# Autodesk Inventor assembly: Electronics V2
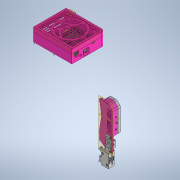
[picture p0: Inventor's stored thumbnail of the model, 180x180]
Saved by Autodesk Inventor 2020.3 (Build 243373010, 373A)
## iProperties
Created: 2019-12-13
Part Number: Electronics V2
Document SubType Name: Assembly
Designer: pepd9
Mass: 362.795 g
Surface Area: 2325.02 cm^2
Volume: 298.236 cm^3
Density: 1.21647 g/cm^3
Author: pepd9
## Documents named in this file (19)
- D:\Designs\MK3PRO P1\ELECTRONICS\Electronics V2.iam
- D:\Designs\MK3PRO P1\COMPONENTS\SHCS_M3_12.ipt
- D:\Designs\MK3PRO P1\COMPONENTS\M3 Nut.ipt
- D:\Designs\MK3PRO P1\ELECTRONICS\LM2596.ipt
- D:\Designs\MK3PRO P1\ELECTRONICS\FAN PS CASE.ipt
- D:\Designs\MK3PRO P1\COMPONENTS\SHCS_M3_8.ipt
- D:\Designs\MK3PRO P1\COMPONENTS\NUT_SQUARE_M3.ipt
- D:\Designs\MK3PRO P1\COMPONENTS\SHCS_M3_10.ipt
- D:\Designs\MK3PRO P1\ELECTRONICS\FAN PS CASE LID.ipt
- D:\Designs\MK3PRO P1\ELECTRONICS\Fan Distribution Case.ipt
- D:\Designs\MK3PRO P1\ELECTRONICS\Double Sided PCB 6x28.iam
- D:\Designs\MK3PRO P1\COMPONENTS\M3 Washer.ipt
- D:\Designs\MK3PRO P1\FRAME\Extruder-Motherboard Cable Clamp.ipt
- D:\Designs\MK3PRO P1\COMPONENTS\SHCS_M3_20.ipt
- D:\Designs\MK3PRO P1\ELECTRONICS\Fan PDP Lid.ipt
- D:\Designs\MK3PRO P1\ELECTRONICS\ID Plate.ipt
- D:\Designs\MK3PRO P1\ELECTRONICS\Rambo Case P1.0.ipt
- D:\Designs\MK3PRO P1\ELECTRONICS\Rambo 1.3.ipt
- D:\Designs\MK3PRO P1\ELECTRONICS\Rambo Case Lid.ipt
## Components (56 placed, 18 different names)
1. LM2596:1 — Mate:14, Mate:15, Mate:18, Mate:19, Mate:20
2. FAN PS CASE:1 — Mate:14, Mate:15, Mate:16, Mate:17, Mate:20, Mate:21, Mate:22, Angle:6, Angle:7, Mate:25, Mate:26, Angle:8, Mate:27, Mate:28, Mate:29, Mate:30, Mate:31, Mate:32, Angle:9
3. SHCS_M3_8:1 — Mate:17, Mate:19, Mate:24
4. SHCS_M3_8:2 — Mate:16, Mate:18, Mate:23
5. M3 Nut:5 — Mate:21, Angle:7, Mate:24
6. M3 Nut:6 — Mate:22, Angle:6, Mate:23
7. NUT_SQUARE_M3:1 — Mate:25, Mate:26, Angle:8
8. SHCS_M3_10:1 — Mate:28, Mate:29
9. SHCS_M3_10:2 — Mate:27, Mate:30
10. SHCS_M3_8:3 — Mate:33, Mate:34
11. FAN PS CASE LID:1 — Mate:31, Mate:32, Angle:9, Mate:33, Mate:34
12. Fan Distribution Case:1 — Mate:35, Angle:10, Mate:36, Mate:37, Mate:42, Mate:44, Mate:47, Mate:56, Mate:57, Mate:58, Mate:59, Angle:11, Angle:12, Mate:64, Mate:65, Mate:66, Mate:67, Mate:72, Mate:73, Mate:74, Mate:75, Angle:15, Angle:16, Mate:76, Mate:77, Mate:84, Angle:17, Mate:86, Angle:18, Mate:138, Mate:139, Mate:140, Mate:142, Mate:147, Flush:1, Mate:149
13. Double Sided PCB 6x28:1 [sub-assembly] — Mate:35, Angle:10, Mate:36, Mate:37
14. Extruder-Motherboard Cable Clamp:2 — Mate:42, Mate:44, Mate:47, Mate:48, Mate:49, Mate:52, Mate:53
15. SHCS_M3_20:2 — Mate:49, Mate:53, Mate:62
16. SHCS_M3_20:4 — Mate:48, Mate:52, Mate:63
17. M3 Nut:7 — Mate:59
18. M3 Nut:8 — Mate:58
19. M3 Nut:9 — Mate:57, Mate:62, Angle:12
20. M3 Nut:10 — Mate:56, Mate:63, Angle:11
21. M3 Nut:11 — Mate:73, Mate:74, Angle:15
22. M3 Nut:12 — Mate:72, Mate:75, Angle:16
23. M3 Washer:2 — Mate:64, Mate:69, Mate:70
24. M3 Washer:3 — Mate:65, Mate:68, Mate:71
25. SHCS_M3_10:4 — Mate:66, Mate:69, Mate:70
26. SHCS_M3_10:5 — Mate:67, Mate:68, Mate:71
27. SHCS_M3_8:4 — Mate:76, Mate:144, Mate:145
28. SHCS_M3_8:5 — Mate:77, Mate:143, Mate:146
29. SHCS_M3_12:3 — Mate:87, Mate:148, Mate:163
30. SHCS_M3_12:4 — Mate:85
31. NUT_SQUARE_M3:2 — Mate:84, Mate:85, Angle:17
32. NUT_SQUARE_M3:3 — Mate:86, Mate:87, Angle:18
33. Rambo Case P1.0:1 — Mate:88, Mate:89, Mate:90, Mate:113, Mate:114, Mate:115, Mate:116, Mate:117, Mate:118, Mate:119, Mate:120, Mate:121, Mate:122, Mate:123, Mate:124, Mate:125, Mate:126, Angle:24, Angle:25, Angle:26, Angle:27, Mate:137, Mate:150, Mate:151, Mate:152, Mate:153, Mate:154, Mate:156, Mate:159, Angle:28
34. Rambo 1.3:1 — Mate:88, Mate:89, Mate:90, Mate:129, Mate:130, Mate:131, Mate:132, Mate:133, Mate:134, Mate:135, Mate:136
35. Rambo Case Lid:1 — Mate:137, Mate:150, Mate:151, Mate:152, Mate:158, Mate:160, Mate:161, Mate:162
36. SHCS_M3_12:5 — Mate:117, Mate:127
37. SHCS_M3_12:6 — Mate:118, Mate:128
38. M3 Washer:4 — Mate:114, Mate:115, Mate:128
39. M3 Washer:5 — Mate:113, Mate:116, Mate:127
40. M3 Nut:13 — Mate:120, Mate:126, Angle:24
41. M3 Nut:14 — Mate:121, Mate:124, Angle:26
42. M3 Nut:15 — Mate:122, Mate:123, Angle:27
43. M3 Nut:16 — Mate:119, Mate:125, Angle:25
44. SHCS_M3_8:6 — Mate:129, Mate:134
45. SHCS_M3_8:7 — Mate:130, Mate:135
46. SHCS_M3_8:8 — Mate:131, Mate:136
47. SHCS_M3_8:9 — Mate:132, Mate:133
48. SHCS_M3_10:6 — Mate:140, Mate:141
49. M3 Washer:6 — Mate:138, Mate:139, Mate:141
50. ID Plate:1 — Mate:142, Mate:143, Mate:144, Mate:145, Mate:146
51. Fan PDP Lid:1 — Mate:147, Mate:148, Flush:1, Mate:149, Mate:163, Mate:164, Mate:165
52. NUT_SQUARE_M3:4 — Mate:156, Mate:159, Angle:28
53. NUT_SQUARE_M3:5 — Mate:153, Mate:154
54. SHCS_M3_10:7 — Mate:158, Mate:160
55. SHCS_M3_10:9 — Mate:161, Mate:162
56. SHCS_M3_12:7 — Mate:164, Mate:165
## Relationships (126: Mate 109, Angle 16, Flush 1)
- Mate:14: LM2596:1 ↔ FAN PS CASE:1
- Mate:15: LM2596:1 ↔ FAN PS CASE:1
- Mate:16: FAN PS CASE:1 ↔ SHCS_M3_8:2
- Mate:17: FAN PS CASE:1 ↔ SHCS_M3_8:1
- Mate:18: LM2596:1 ↔ SHCS_M3_8:2
- Mate:19: LM2596:1 ↔ SHCS_M3_8:1
- Mate:20: LM2596:1 ↔ FAN PS CASE:1
- Mate:21: FAN PS CASE:1 ↔ M3 Nut:5
- Mate:22: FAN PS CASE:1 ↔ M3 Nut:6
- Angle:6 (0 deg): FAN PS CASE:1 ↔ M3 Nut:6
- Mate:23: SHCS_M3_8:2 ↔ M3 Nut:6
- Angle:7 (0 deg): FAN PS CASE:1 ↔ M3 Nut:5
- Mate:24: SHCS_M3_8:1 ↔ M3 Nut:5
- Mate:25: FAN PS CASE:1 ↔ NUT_SQUARE_M3:1
- Mate:26: FAN PS CASE:1 ↔ NUT_SQUARE_M3:1
- Angle:8 (0 deg): FAN PS CASE:1 ↔ NUT_SQUARE_M3:1
- Mate:27: FAN PS CASE:1 ↔ SHCS_M3_10:2
- Mate:28: FAN PS CASE:1 ↔ SHCS_M3_10:1
- Mate:29: FAN PS CASE:1 ↔ SHCS_M3_10:1
- Mate:30: FAN PS CASE:1 ↔ SHCS_M3_10:2
- Mate:31: FAN PS CASE:1 ↔ FAN PS CASE LID:1
- Mate:32: FAN PS CASE:1 ↔ FAN PS CASE LID:1
- Angle:9 (180 deg): FAN PS CASE:1 ↔ FAN PS CASE LID:1
- Mate:33: SHCS_M3_8:3 ↔ FAN PS CASE LID:1
- Mate:34: SHCS_M3_8:3 ↔ FAN PS CASE LID:1
- Mate:35: Fan Distribution Case:1 ↔ Double Sided PCB 6x28:1
- Angle:10 (0 deg): Fan Distribution Case:1 ↔ Double Sided PCB 6x28:1
- Mate:36 (-40 mm): Fan Distribution Case:1 ↔ Double Sided PCB 6x28:1
- Mate:37 (0.3 mm): Fan Distribution Case:1 ↔ Double Sided PCB 6x28:1
- Mate:42: Fan Distribution Case:1 ↔ Extruder-Motherboard Cable Clamp:2
- Mate:44: Fan Distribution Case:1 ↔ Extruder-Motherboard Cable Clamp:2
- Mate:47: Fan Distribution Case:1 ↔ Extruder-Motherboard Cable Clamp:2
- Mate:48: Extruder-Motherboard Cable Clamp:2 ↔ SHCS_M3_20:4
- Mate:49: Extruder-Motherboard Cable Clamp:2 ↔ SHCS_M3_20:2
- Mate:52: Extruder-Motherboard Cable Clamp:2 ↔ SHCS_M3_20:4
- Mate:53: Extruder-Motherboard Cable Clamp:2 ↔ SHCS_M3_20:2
- Mate:56: Fan Distribution Case:1 ↔ M3 Nut:10
- Mate:57: Fan Distribution Case:1 ↔ M3 Nut:9
- Mate:58: Fan Distribution Case:1 ↔ M3 Nut:8
- Mate:59: Fan Distribution Case:1 ↔ M3 Nut:7
- Mate:62: SHCS_M3_20:2 ↔ M3 Nut:9
- Mate:63: SHCS_M3_20:4 ↔ M3 Nut:10
- Angle:11 (0 deg): Fan Distribution Case:1 ↔ M3 Nut:10
- Angle:12 (0 deg): Fan Distribution Case:1 ↔ M3 Nut:9
- Mate:64: Fan Distribution Case:1 ↔ M3 Washer:2
- Mate:65: Fan Distribution Case:1 ↔ M3 Washer:3
- Mate:66: Fan Distribution Case:1 ↔ SHCS_M3_10:4
- Mate:67: Fan Distribution Case:1 ↔ SHCS_M3_10:5
- Mate:68: M3 Washer:3 ↔ SHCS_M3_10:5
- Mate:69: M3 Washer:2 ↔ SHCS_M3_10:4
- Mate:70: M3 Washer:2 ↔ SHCS_M3_10:4
- Mate:71: M3 Washer:3 ↔ SHCS_M3_10:5
- Mate:72: Fan Distribution Case:1 ↔ M3 Nut:12
- Mate:73: Fan Distribution Case:1 ↔ M3 Nut:11
- Mate:74: Fan Distribution Case:1 ↔ M3 Nut:11
- Mate:75: Fan Distribution Case:1 ↔ M3 Nut:12
- Angle:15 (0 deg): Fan Distribution Case:1 ↔ M3 Nut:11
- Angle:16 (0 deg): Fan Distribution Case:1 ↔ M3 Nut:12
- Mate:76: Fan Distribution Case:1 ↔ SHCS_M3_8:4
- Mate:77: Fan Distribution Case:1 ↔ SHCS_M3_8:5
- Mate:84: Fan Distribution Case:1 ↔ NUT_SQUARE_M3:2
- Mate:85: SHCS_M3_12:4 ↔ NUT_SQUARE_M3:2
- Angle:17 (0 deg): Fan Distribution Case:1 ↔ NUT_SQUARE_M3:2
- Mate:86: Fan Distribution Case:1 ↔ NUT_SQUARE_M3:3
- Mate:87: SHCS_M3_12:3 ↔ NUT_SQUARE_M3:3
- Angle:18 (0 deg): Fan Distribution Case:1 ↔ NUT_SQUARE_M3:3
- Mate:88: Rambo Case P1.0:1 ↔ Rambo 1.3:1
- Mate:89: Rambo Case P1.0:1 ↔ Rambo 1.3:1
- Mate:90: Rambo Case P1.0:1 ↔ Rambo 1.3:1
- Mate:113: Rambo Case P1.0:1 ↔ M3 Washer:5
- Mate:114: Rambo Case P1.0:1 ↔ M3 Washer:4
- Mate:115: Rambo Case P1.0:1 ↔ M3 Washer:4
- Mate:116: Rambo Case P1.0:1 ↔ M3 Washer:5
- Mate:117: Rambo Case P1.0:1 ↔ SHCS_M3_12:5
- Mate:118: Rambo Case P1.0:1 ↔ SHCS_M3_12:6
- Mate:119: Rambo Case P1.0:1 ↔ M3 Nut:16
- Mate:120: Rambo Case P1.0:1 ↔ M3 Nut:13
- Mate:121: Rambo Case P1.0:1 ↔ M3 Nut:14
- Mate:122: Rambo Case P1.0:1 ↔ M3 Nut:15
- Mate:123: Rambo Case P1.0:1 ↔ M3 Nut:15
- Mate:124: Rambo Case P1.0:1 ↔ M3 Nut:14
- Mate:125: Rambo Case P1.0:1 ↔ M3 Nut:16
- Mate:126: Rambo Case P1.0:1 ↔ M3 Nut:13
- Angle:24 (0 deg): Rambo Case P1.0:1 ↔ M3 Nut:13
- Angle:25 (0 deg): Rambo Case P1.0:1 ↔ M3 Nut:16
- Angle:26 (0 deg): Rambo Case P1.0:1 ↔ M3 Nut:14
- Angle:27 (0 deg): Rambo Case P1.0:1 ↔ M3 Nut:15
- Mate:127: SHCS_M3_12:5 ↔ M3 Washer:5
- Mate:128: SHCS_M3_12:6 ↔ M3 Washer:4
- Mate:129: Rambo 1.3:1 ↔ SHCS_M3_8:6
- Mate:130: Rambo 1.3:1 ↔ SHCS_M3_8:7
- Mate:131: Rambo 1.3:1 ↔ SHCS_M3_8:8
- Mate:132: Rambo 1.3:1 ↔ SHCS_M3_8:9
- Mate:133: Rambo 1.3:1 ↔ SHCS_M3_8:9
- Mate:134: Rambo 1.3:1 ↔ SHCS_M3_8:6
- Mate:135: Rambo 1.3:1 ↔ SHCS_M3_8:7
- Mate:136: Rambo 1.3:1 ↔ SHCS_M3_8:8
- Mate:137: Rambo Case P1.0:1 ↔ Rambo Case Lid:1
- Mate:138: Fan Distribution Case:1 ↔ M3 Washer:6
- Mate:139: Fan Distribution Case:1 ↔ M3 Washer:6
- Mate:140: Fan Distribution Case:1 ↔ SHCS_M3_10:6
- Mate:141: SHCS_M3_10:6 ↔ M3 Washer:6
- Mate:142: Fan Distribution Case:1 ↔ ID Plate:1
- Mate:143: SHCS_M3_8:5 ↔ ID Plate:1
- Mate:144: SHCS_M3_8:4 ↔ ID Plate:1
- Mate:145: SHCS_M3_8:4 ↔ ID Plate:1
- Mate:146: SHCS_M3_8:5 ↔ ID Plate:1
- Mate:147: Fan Distribution Case:1 ↔ Fan PDP Lid:1
- Mate:148: SHCS_M3_12:3 ↔ Fan PDP Lid:1
- Flush:1: Fan Distribution Case:1 ↔ Fan PDP Lid:1
- Mate:149: Fan Distribution Case:1 ↔ Fan PDP Lid:1
- Mate:150: Rambo Case P1.0:1 ↔ Rambo Case Lid:1
- Mate:151: Rambo Case P1.0:1 ↔ Rambo Case Lid:1
- Mate:152: Rambo Case P1.0:1 ↔ Rambo Case Lid:1
- Mate:153: Rambo Case P1.0:1 ↔ NUT_SQUARE_M3:5
- Mate:154: Rambo Case P1.0:1 ↔ NUT_SQUARE_M3:5
- Mate:156: Rambo Case P1.0:1 ↔ NUT_SQUARE_M3:4
- Mate:158: Rambo Case Lid:1 ↔ SHCS_M3_10:7
- Mate:159: Rambo Case P1.0:1 ↔ NUT_SQUARE_M3:4
- Angle:28 (0 deg): Rambo Case P1.0:1 ↔ NUT_SQUARE_M3:4
- Mate:160: Rambo Case Lid:1 ↔ SHCS_M3_10:7
- Mate:161: Rambo Case Lid:1 ↔ SHCS_M3_10:9
- Mate:162: Rambo Case Lid:1 ↔ SHCS_M3_10:9
- Mate:163: SHCS_M3_12:3 ↔ Fan PDP Lid:1
- Mate:164: Fan PDP Lid:1 ↔ SHCS_M3_12:7
- Mate:165: Fan PDP Lid:1 ↔ SHCS_M3_12:7
